# Autodesk Inventor assembly: RCR_drive
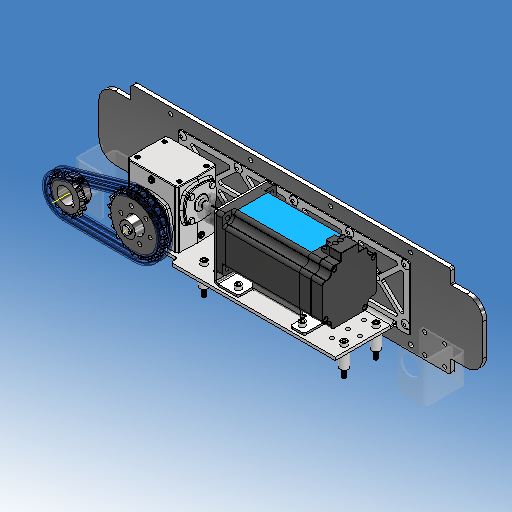
[picture p0: Inventor's stored thumbnail of the model, 512x512]
Saved by Autodesk Inventor 2025 (Build 290162000, 162)
## iProperties
Created: 2024-02-27
Part Number: RCR_drive
Document SubType Name: Assembly
Designer: seene
Author: seene
## Documents named in this file (20)
- C:\Users\seene\Desktop\Stony Brook\SBRT\RCR_Dexter\Drive\RCR_drive -flipped.iam
- C:\Users\seene\Desktop\Stony Brook\SBRT\RCR_Dexter\Drive\v1\ChassisInterface.ipt
- C:\Users\seene\Desktop\Stony Brook\SBRT\RCR_Dexter\Drive\v1\2299K28_Flat Sprocket.ipt
- C:\Users\seene\Desktop\Stony Brook\SBRT\RCR_Dexter\Drive\v1\9939T12_Durometer 64D Spider for 1-5 16 OD Set Screw Vibrate-Damping Precision Flexible Shaft Coupling.ipt
- C:\Users\seene\Desktop\Stony Brook\SBRT\RCR_Dexter\Drive\v1\9939T102_Vibrate-Damping Precision Flexible Shaft Coupling.ipt
- C:\Users\seene\Desktop\Stony Brook\SBRT\RCR_Dexter\Drive\v1\9939T104_Vibrate-Damping Precision Flexible Shaft Coupling.ipt
- C:\Users\seene\Desktop\Stony Brook\SBRT\RCR_Dexter\Drive\v1\am-0077a 500 Key Hub REV3.ipt
- C:\Users\seene\Desktop\Stony Brook\SBRT\RCR_Dexter\Drive\v1\6280K675_Roller Chain Sprocket.ipt
- C:\Users\seene\Desktop\Stony Brook\SBRT\RCR_Dexter\Drive\v1\40 chain link.ipt
- C:\Users\seene\Desktop\Stony Brook\SBRT\RCR_Dexter\Drive\v1\34HS59-6004D-E1000 .ipt
- C:\Users\seene\Desktop\Stony Brook\SBRT\RCR_Dexter\Drive\v1\StepperMotorStandOff.ipt
- C:\Users\seene\Desktop\Stony Brook\SBRT\RCR_Dexter\Drive\v1\DriveShaftSupport.ipt
- C:\Users\seene\Desktop\Stony Brook\SBRT\RCR_Dexter\Drive\v1\DriveShaftSupport _Flipped.ipt
- C:\Users\seene\Desktop\Stony Brook\SBRT\RCR_Dexter\Drive\QuintinCAD\Flipped_MainDriveMount.ipt
- C:\Users\seene\Desktop\Stony Brook\SBRT\RCR_Dexter\Drive\v1\5887K171_Right-Angle Speed Reducer.ipt
- C:\Users\seene\Desktop\Stony Brook\SBRT\RCR_Dexter\Drive\RCR_drive -flipped\Design Accelerator\Chain Drive2.iam
- C:\Users\seene\Desktop\Stony Brook\SBRT\RCR_Dexter\Drive\v1\DriveMountStandoff.ipt
- C:\Users\seene\Desktop\Stony Brook\SBRT\RCR_Dexter\Drive\v1\90128A252_Zinc-Plated Alloy Steel Socket Head Screw.ipt
- C:\Users\seene\Desktop\Stony Brook\SBRT\RCR_Dexter\Drive\v1\97525A550_18-8 Stainless Steel Blind Rivets.ipt
- C:\Users\seene\Desktop\Stony Brook\SBRT\RCR_Dexter\Drive\v1\91274A156_Zinc-Aluminum-Coated Alloy Steel Socket Head Screw.ipt
## Components (44 placed, 19 different names)
1. 2299K28_Flat Sprocket:1 — Mate:23, Mate:24, Mate:25, Flush:7, Mate:133, Mate:134, Mate:135, Mate:136, Mate:137, Flush:46, Mate:329
2. 9939T12_Durometer 64D Spider for 1-5 16 OD Set Screw Vibrate-Damping Precision Flexible Shaft Coupling:1 — Mate:1, Mate:7, Mate:8, Mate:9
3. 9939T102_Vibrate-Damping Precision Flexible Shaft Coupling:1 — Mate:8, Mate:9, Mate:330
4. 9939T104_Vibrate-Damping Precision Flexible Shaft Coupling:1 — Mate:1, Mate:7
5. am-0077a 500 Key Hub REV3:1 — Mate:23, Mate:24, Mate:25, Mate:327, Mate:328
6. 6280K675_Roller Chain Sprocket:1 — Flush:7, Flush:46, Mate:336
7. 34HS59-6004D-E1000 :1 — Mate:251, Flush:45, Mate:255, Mate:256, Mate:257
8. ChassisInterface:2 — Mate:287, Mate:309, Mate:319, Mate:320, Mate:321, Mate:332, Mate:333, Mate:334, Mate:335
9. StepperMotorStandOff:1 — Mate:251, Flush:45, Mate:255, Mate:256, Mate:257, Mate:322, Mate:323, Mate:324, Mate:345, Mate:346
10. DriveShaftSupport:1 — Mate:287, Mate:332, Mate:335, Mate:336
11. DriveShaftSupport _Flipped:1 — Mate:309, Mate:333, Mate:334
12. Flipped_MainDriveMount:1 — Mate:319, Mate:320, Mate:321, Mate:322, Mate:323, Mate:324, Mate:326, Mate:331, Mate:337, Mate:339, Mate:341, Mate:342, Mate:343, Mate:344, Mate:347
13. 5887K171_Right-Angle Speed Reducer:1 — Mate:326, Mate:327, Mate:328, Mate:330, Mate:331
14. Chain Drive:2 [sub-assembly]
15. 40 chain link:1 — Mate:127, Mate:130, Mate:136, Mate:137
16. 40 chain link:2 — Mate:129, Mate:132, Mate:135, Mate:329
17. 40 chain link:3 — Mate:128, Mate:129, Mate:131, Mate:132, Mate:134
18. 40 chain link:4 — Mate:127, Mate:128, Mate:130, Mate:131, Mate:133
19. DriveMountStandoff:4 — Mate:337, Mate:339, Mate:340
20. 90128A252_Zinc-Plated Alloy Steel Socket Head Screw:1 — Mate:340, Mate:341
21. DriveMountStandoff:5
22. 90128A252_Zinc-Plated Alloy Steel Socket Head Screw:2
23. DriveMountStandoff:6
24. 90128A252_Zinc-Plated Alloy Steel Socket Head Screw:3
25. DriveMountStandoff:7
26. 90128A252_Zinc-Plated Alloy Steel Socket Head Screw:4
27. 97525A550_18-8 Stainless Steel Blind Rivets:1 — Mate:342, Mate:343
28. 97525A550_18-8 Stainless Steel Blind Rivets:2
29. 97525A550_18-8 Stainless Steel Blind Rivets:3
30. 97525A550_18-8 Stainless Steel Blind Rivets:4
31. 97525A550_18-8 Stainless Steel Blind Rivets:5
32. 97525A550_18-8 Stainless Steel Blind Rivets:6
33. 97525A550_18-8 Stainless Steel Blind Rivets:7
34. 97525A550_18-8 Stainless Steel Blind Rivets:8
35. 97525A550_18-8 Stainless Steel Blind Rivets:9
36. 97525A550_18-8 Stainless Steel Blind Rivets:10
37. 91274A156_Zinc-Aluminum-Coated Alloy Steel Socket Head Screw:2 — Mate:345, Mate:346
38. 91274A156_Zinc-Aluminum-Coated Alloy Steel Socket Head Screw:3
39. 91274A156_Zinc-Aluminum-Coated Alloy Steel Socket Head Screw:4
40. 91274A156_Zinc-Aluminum-Coated Alloy Steel Socket Head Screw:5
41. 91274A156_Zinc-Aluminum-Coated Alloy Steel Socket Head Screw:1 — Mate:344, Mate:347
42. 91274A156_Zinc-Aluminum-Coated Alloy Steel Socket Head Screw:6
43. 91274A156_Zinc-Aluminum-Coated Alloy Steel Socket Head Screw:7
44. 91274A156_Zinc-Aluminum-Coated Alloy Steel Socket Head Screw:8
## Component patterns: (4 elements, first: DriveMountStandoff:4 + 90128A252_Zinc-Plated Alloy Steel Socket Head Screw:1), (10 elements, first: 97525A550_18-8 Stainless Steel Blind Rivets:1), (4 elements, first: 91274A156_Zinc-Aluminum-Coated Alloy Steel Socket Head Screw:2), (4 elements, first: 91274A156_Zinc-Aluminum-Coated Alloy Steel Socket Head Screw:1)
## Relationships (54: Mate 51, Flush 3)
- Mate:1: 9939T12_Durometer 64D Spider for 1-5 16 OD Set Screw Vibrate-Damping Precision Flexible Shaft Coupling:1 ↔ 9939T104_Vibrate-Damping Precision Flexible Shaft Coupling:1
- Mate:7: 9939T12_Durometer 64D Spider for 1-5 16 OD Set Screw Vibrate-Damping Precision Flexible Shaft Coupling:1 ↔ 9939T104_Vibrate-Damping Precision Flexible Shaft Coupling:1
- Mate:8: 9939T12_Durometer 64D Spider for 1-5 16 OD Set Screw Vibrate-Damping Precision Flexible Shaft Coupling:1 ↔ 9939T102_Vibrate-Damping Precision Flexible Shaft Coupling:1
- Mate:9: 9939T12_Durometer 64D Spider for 1-5 16 OD Set Screw Vibrate-Damping Precision Flexible Shaft Coupling:1 ↔ 9939T102_Vibrate-Damping Precision Flexible Shaft Coupling:1
- Mate:23: 2299K28_Flat Sprocket:1 ↔ am-0077a 500 Key Hub REV3:1
- Mate:24: 2299K28_Flat Sprocket:1 ↔ am-0077a 500 Key Hub REV3:1
- Mate:25: 2299K28_Flat Sprocket:1 ↔ am-0077a 500 Key Hub REV3:1
- Flush:7: 2299K28_Flat Sprocket:1 ↔ 6280K675_Roller Chain Sprocket:1
- Mate:127: 40 chain link:1 ↔ 40 chain link:4
- Mate:128: 40 chain link:3 ↔ 40 chain link:4
- Mate:129: 40 chain link:2 ↔ 40 chain link:3
- Mate:130: 40 chain link:1 ↔ 40 chain link:4
- Mate:131: 40 chain link:3 ↔ 40 chain link:4
- Mate:132: 40 chain link:2 ↔ 40 chain link:3
- Mate:133: 2299K28_Flat Sprocket:1 ↔ 40 chain link:4
- Mate:134: 2299K28_Flat Sprocket:1 ↔ 40 chain link:3
- Mate:135: 2299K28_Flat Sprocket:1 ↔ 40 chain link:2
- Mate:136: 2299K28_Flat Sprocket:1 ↔ 40 chain link:1
- Mate:137: 2299K28_Flat Sprocket:1 ↔ 40 chain link:1
- Mate:251: 34HS59-6004D-E1000 :1 ↔ StepperMotorStandOff:1
- Flush:45: 34HS59-6004D-E1000 :1 ↔ StepperMotorStandOff:1
- Mate:255: 34HS59-6004D-E1000 :1 ↔ StepperMotorStandOff:1
- Mate:256: 34HS59-6004D-E1000 :1 ↔ StepperMotorStandOff:1
- Mate:257: 34HS59-6004D-E1000 :1 ↔ StepperMotorStandOff:1
- Mate:287: ChassisInterface:2 ↔ DriveShaftSupport:1
- Mate:309: ChassisInterface:2 ↔ DriveShaftSupport _Flipped:1
- Flush:46: 2299K28_Flat Sprocket:1 ↔ 6280K675_Roller Chain Sprocket:1
- Mate:319: ChassisInterface:2 ↔ Flipped_MainDriveMount:1
- Mate:320: ChassisInterface:2 ↔ Flipped_MainDriveMount:1
- Mate:321: ChassisInterface:2 ↔ Flipped_MainDriveMount:1
- Mate:322: StepperMotorStandOff:1 ↔ Flipped_MainDriveMount:1
- Mate:323: StepperMotorStandOff:1 ↔ Flipped_MainDriveMount:1
- Mate:324: StepperMotorStandOff:1 ↔ Flipped_MainDriveMount:1
- Mate:326: Flipped_MainDriveMount:1 ↔ 5887K171_Right-Angle Speed Reducer:1
- Mate:327: am-0077a 500 Key Hub REV3:1 ↔ 5887K171_Right-Angle Speed Reducer:1
- Mate:328 (3.175 mm): am-0077a 500 Key Hub REV3:1 ↔ 5887K171_Right-Angle Speed Reducer:1
- Mate:329: 2299K28_Flat Sprocket:1 ↔ 40 chain link:2
- Mate:330: 9939T102_Vibrate-Damping Precision Flexible Shaft Coupling:1 ↔ 5887K171_Right-Angle Speed Reducer:1
- Mate:331: Flipped_MainDriveMount:1 ↔ 5887K171_Right-Angle Speed Reducer:1
- Mate:332: ChassisInterface:2 ↔ DriveShaftSupport:1
- Mate:333: ChassisInterface:2 ↔ DriveShaftSupport _Flipped:1
- Mate:334: ChassisInterface:2 ↔ DriveShaftSupport _Flipped:1
- Mate:335: ChassisInterface:2 ↔ DriveShaftSupport:1
- Mate:336: 6280K675_Roller Chain Sprocket:1 ↔ DriveShaftSupport:1
- Mate:337: Flipped_MainDriveMount:1 ↔ DriveMountStandoff:4
- Mate:339: Flipped_MainDriveMount:1 ↔ DriveMountStandoff:4
- Mate:340: DriveMountStandoff:4 ↔ 90128A252_Zinc-Plated Alloy Steel Socket Head Screw:1
- Mate:341: Flipped_MainDriveMount:1 ↔ 90128A252_Zinc-Plated Alloy Steel Socket Head Screw:1
- Mate:342: Flipped_MainDriveMount:1 ↔ 97525A550_18-8 Stainless Steel Blind Rivets:1
- Mate:343: Flipped_MainDriveMount:1 ↔ 97525A550_18-8 Stainless Steel Blind Rivets:1
- Mate:344: Flipped_MainDriveMount:1 ↔ 91274A156_Zinc-Aluminum-Coated Alloy Steel Socket Head Screw:1
- Mate:345: StepperMotorStandOff:1 ↔ 91274A156_Zinc-Aluminum-Coated Alloy Steel Socket Head Screw:2
- Mate:346: StepperMotorStandOff:1 ↔ 91274A156_Zinc-Aluminum-Coated Alloy Steel Socket Head Screw:2
- Mate:347: Flipped_MainDriveMount:1 ↔ 91274A156_Zinc-Aluminum-Coated Alloy Steel Socket Head Screw:1
